# Autodesk Inventor assembly: modular predator mount
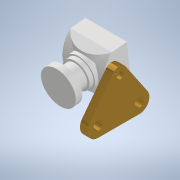
[picture p0: Inventor's stored thumbnail of the model, 180x180]
Saved by Autodesk Inventor 2020 (Build 240168000, 168)
## iProperties
Created: 2022-05-05
Part Number: modular predator mount
Document SubType Name: Assembly
Designer: Steven
Author: Steven
## Documents named in this file (3)
- Y:\FPV drone stuff\0 Street League\Frames\PB-Kauri-X\3D prints\35 mm canopy\work in progress prints\modular predator mount.iam
- Y:\FPV drone stuff\0 Street League\Frames\PB-Kauri-X\3D prints\35 mm canopy\work in progress prints\mini predator dummy camera.ipt
- Y:\FPV drone stuff\0 Street League\Frames\PB-Kauri-X\3D prints\35 mm canopy\work in progress prints\Kauri modular camera mount mini.ipt
## Components (2 placed, 2 different names)
1. mini predator dummy camera:1 — Insert:1
2. Kauri modular camera mount mini:1 — Insert:1, Mate:1
## Relationships (2: Insert 1, Mate 1)
- Insert:1: mini predator dummy camera:1 ↔ Kauri modular camera mount mini:1
- Mate:1: Kauri modular camera mount mini:1
